# Autodesk Inventor assembly: RemoteCameraModule
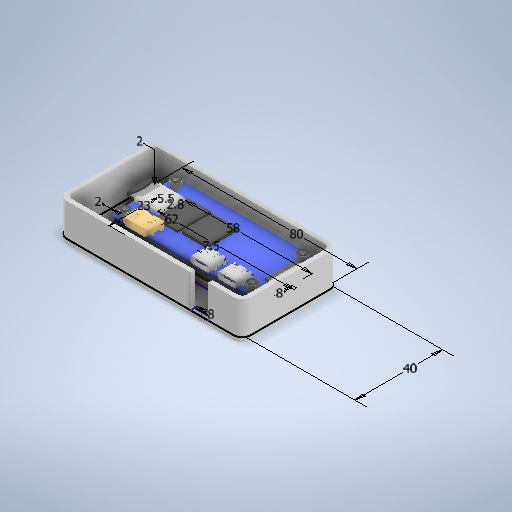
[picture p0: Inventor's stored thumbnail of the model, 512x512]
Saved by Autodesk Inventor 2025 (Build 290162000, 162)
## iProperties
Created: 2025-02-27
Part Number: RemoteCameraModule
Document SubType Name: Assembly
Designer: tvoko
Author: tvoko
## Documents named in this file (5)
- D:\github\enhanced-radio-comm\demo-hardware\RemoteCameraModule.iam
- C:\Users\tvoko\Documents\School\Fall 2024\Senior Design Pt 1\Lab 1\Buyouts\OPiZ2W_\OPiZ2W_.ipt
- D:\github\enhanced-radio-comm\demo-hardware\PiMountBracket.ipt
- C:\Users\tvoko\Documents\Inventor\Content Center Files\R2025\en-US\IS 2269\IS 2269 - M2.5 x 8.ipt
- D:\github\enhanced-radio-comm\demo-hardware\RemoteCasing.ipt
## Components (7 placed, 4 different names)
1. OPiZ2W_:1 — Mate:1, Mate:2, Mate:3, Mate:8, Mate:10, Mate:12, Mate:14
2. PiMountBracket:1 — Mate:1, Mate:2, Mate:3, Mate:4, Mate:9, Mate:11, Mate:13
3. IS 2269 M2.5 x 8:1 — Mate:4, Mate:8, Mate:15, Mate:17
4. IS 2269 M2.5 x 8:2 — Mate:9, Mate:10
5. IS 2269 M2.5 x 8:3 — Mate:11, Mate:12, Mate:16
6. IS 2269 M2.5 x 8:4 — Mate:13, Mate:14
7. RemoteCasing:1 — Mate:15, Mate:16, Mate:17
## Relationships (14: Mate 14)
- Mate:1: OPiZ2W_:1 ↔ PiMountBracket:1
- Mate:2: OPiZ2W_:1 ↔ PiMountBracket:1
- Mate:3: OPiZ2W_:1 ↔ PiMountBracket:1
- Mate:4: PiMountBracket:1 ↔ IS 2269 M2.5 x 8:1
- Mate:8: OPiZ2W_:1 ↔ IS 2269 M2.5 x 8:1
- Mate:9: PiMountBracket:1 ↔ IS 2269 M2.5 x 8:2
- Mate:10: OPiZ2W_:1 ↔ IS 2269 M2.5 x 8:2
- Mate:11: PiMountBracket:1 ↔ IS 2269 M2.5 x 8:3
- Mate:12: OPiZ2W_:1 ↔ IS 2269 M2.5 x 8:3
- Mate:13: PiMountBracket:1 ↔ IS 2269 M2.5 x 8:4
- Mate:14: OPiZ2W_:1 ↔ IS 2269 M2.5 x 8:4
- Mate:15: IS 2269 M2.5 x 8:1 ↔ RemoteCasing:1
- Mate:16: IS 2269 M2.5 x 8:3 ↔ RemoteCasing:1
- Mate:17: IS 2269 M2.5 x 8:1 ↔ RemoteCasing:1
